# Autodesk Inventor assembly: BallRotatorMachine
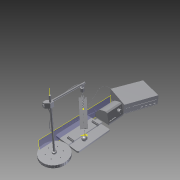
[picture p0: Inventor's stored thumbnail of the model, 180x180]
Saved by Autodesk Inventor 2012 SP2 (Build 160219200, 219)
## iProperties
Created: 2014-02-06
Part Number: BallRotatorMachine
Document SubType Name: Assembly
Designer: 1
Author: 1
## Documents named in this file (13)
- D:\p3_metod1580library\figures\sources\M7-BallRotatorMachine\BallRotatorMachine.iam
- D:\p3_metod1580library\figures\sources\M7-BallRotatorMachine\Stand.ipt
- D:\p3_metod1580library\figures\sources\M7-BallRotatorMachine\MotorCarrier.ipt
- D:\p3_metod1580library\figures\sources\M7-BallRotatorMachine\HorStrut.ipt
- D:\p3_metod1580library\figures\sources\M7-BallRotatorMachine\MotorHolder.ipt
- D:\p3_metod1580library\figures\sources\M7-BallRotatorMachine\Bolt1.ipt
- D:\p3_metod1580library\figures\sources\M7-BallRotatorMachine\Motor.ipt
- D:\p3_metod1580library\figures\sources\M7-BallRotatorMachine\ForceMeterAsmy.iam
- D:\p3_metod1580library\figures\sources\M7-BallRotatorMachine\Ruler.ipt
- D:\p3_metod1580library\figures\sources\M7-BallRotatorMachine\VoltageSource.ipt
- D:\p3_metod1580library\figures\sources\M1-AtwoodsMachine\AbstractBox.ipt
- D:\p3_metod1580library\figures\sources\M7-BallRotatorMachine\Wire1.ipt
- D:\p3_metod1580library\figures\sources\M7-BallRotatorMachine\Wire2.ipt
## Components (13 placed, 12 different names)
1. Stand:1 — Flush:1, Tangent:1
2. MotorCarrier:1 — Flush:2
3. HorStrut:1 — Flush:2, Tangent:2
4. MotorHolder:1 — Flush:3, Mate:1, Mate:2, Flush:4
5. Bolt1:1 — Flush:3
6. Bolt1:2 — Mate:1, Mate:2
7. Motor:1 — Flush:4
8. ForceMeterAsmy:1 [sub-assembly]
9. Ruler:1 — Flush:5
10. VoltageSource:1 — Flush:6, Flush:7
11. AbstractBox:1 — Mate:3, Flush:8
12. Wire1:1 — Flush:7
13. Wire2:1 — Flush:8
## Relationships (15: Flush 8, Mate 3, Angle 2, Tangent 2)
- Flush:1: Stand:1
- Angle:1 (0 deg)
- Tangent:1: Stand:1
- Flush:2: MotorCarrier:1 ↔ HorStrut:1
- Angle:2 (0 deg)
- Tangent:2: HorStrut:1
- Flush:3: MotorHolder:1 ↔ Bolt1:1
- Mate:1: MotorHolder:1 ↔ Bolt1:2
- Mate:2: MotorHolder:1 ↔ Bolt1:2
- Flush:4: MotorHolder:1 ↔ Motor:1
- Flush:5: Ruler:1
- Flush:6: VoltageSource:1
- Mate:3: AbstractBox:1
- Flush:7: VoltageSource:1 ↔ Wire1:1
- Flush:8: AbstractBox:1 ↔ Wire2:1
